# Autodesk Inventor assembly: EnsambleTuberiaVacio-Desfogue-Condensados
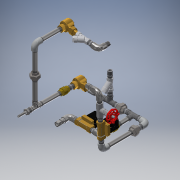
[picture p0: Inventor's stored thumbnail of the model, 180x180]
Saved by Autodesk Inventor 2017 (Build 210142000, 142)
## iProperties
Created: 2021-06-28
Part Number: EnsambleTuberiaVacio-Desfogue-Condensados
Document SubType Name: Assembly
Designer: USUARIO
Author: USUARIO
## Documents named in this file (17)
- D:\Laboratorio\Autoclave\Autoclave Horizontal\Con Precamara\2021\Autoclave 110L Biocacol OP2021110 #0045886XX\Modelo\Planos\EnsambleTuberiaVacio-Desfogue-Condensados.iam
- C:\Modelos 3D y DXF\Filtro en Y\Filtro Y 1-2'' Inox.ipt
- C:\Modelos 3D y DXF\Racores\B122 1-2x1-2.ipt
- C:\Modelos 3D y DXF\Racores\User Library-Tee_Class300.ipt
- C:\Modelos 3D y DXF\Racores\TRAMPA SPIRAX SARCO.ipt
- C:\Modelos 3D y DXF\Racores\Universal1-2.ipt
- C:\Modelos 3D y DXF\Racores\Niple 1-2x3.ipt
- C:\Modelos 3D y DXF\Racores\Check Valve 0.5.ipt
- C:\Modelos 3D y DXF\Racores\CodoCalle.iam
- C:\Modelos 3D y DXF\Danfoss EV210B\DANFOS EV225B.ipt
- C:\Modelos 3D y DXF\Racores\1-2-1-2-SwagelokCompany-3D-06-16-2021.ipt
- C:\Modelos 3D y DXF\Racores\User Library-codo a 90 de 1-2-Rosc.ipt
- C:\Modelos 3D y DXF\Racores\Niple 1-2x6.ipt
- D:\Laboratorio\Autoclave\Autoclave Horizontal\Con Precamara\2021\Autoclave 110L Biocacol OP2021110 #0045886XX\Modelo\UNION LISA 1-2.ipt
- C:\Modelos 3D y DXF\Racores\Niple 1-2x5.ipt
- C:\Modelos 3D y DXF\Racores\B3 1-2x1-2.ipt
- C:\Modelos 3D y DXF\Valvula de Globo\458513-15.iam
## Components (44 placed, 16 different names)
1. Filtro Y 1-2'' Inox:1
2. B122 1-2x1-2:1
3. B122 1-2x1-2:2
4. User Library-Tee_Class300:1
5. TRAMPA SPIRAX SARCO:1
6. B122 1-2x1-2:3
7. Universal1-2:1
8. B122 1-2x1-2:4
9. User Library-Tee_Class300:2
10. Niple 1-2x3:1
11. Check Valve 0.5:1
12. CodoCalle:1 [sub-assembly]
13. B122 1-2x1-2:5
14. DANFOS EV225B:1
15. CodoCalle:2 [sub-assembly]
16. 1-2-1-2-SwagelokCompany-3D-06-16-2021:1
17. User Library-codo a 90 de 1-2-Rosc:1
18. B122 1-2x1-2:6
19. User Library-codo a 90 de 1-2-Rosc:2
20. B122 1-2x1-2:7
21. Universal1-2:2
22. Niple 1-2x6:1
23. B122 1-2x1-2:8
24. DANFOS EV225B:2
25. B122 1-2x1-2:9
26. Check Valve 0.5:2
27. Filtro Y 1-2'' Inox:2
28. B122 1-2x1-2:10
29. CodoCalle:3 [sub-assembly]
30. TRAMPA SPIRAX SARCO:2
31. UNION LISA 1-2:1
32. Niple 1-2x3:2
33. Niple 1-2x5:1
34. Niple 1-2x5:2
35. User Library-codo a 90 de 1-2-Rosc:3
36. User Library-Tee_Class300:3
37. Universal1-2:3
38. Niple 1-2x5:3
39. Niple 1-2x5:4
40. B3 1-2x1-2:1
41. 458513-15:1 [sub-assembly]
42. B122 1-2x1-2:11
43. 1-2-1-2-SwagelokCompany-3D-06-16-2021:2
44. CodoCalle:4 [sub-assembly]
## Relationships (42: Insert 42)
- [Insert] (7 mm): Filtro Y 1-2'' Inox:1 ↔ B122 1-2x1-2:1
- [Insert] (9 mm): B122 1-2x1-2:2 ↔ User Library-Tee_Class300:1
- [Insert] (-7 mm): Filtro Y 1-2'' Inox:1 ↔ B122 1-2x1-2:2
- [Insert] (-9 mm): User Library-Tee_Class300:1 ↔ B122 1-2x1-2:3
- [Insert] (-12 mm): B122 1-2x1-2:3 ↔ Universal1-2:1
- [Insert] (-12 mm): Universal1-2:1 ↔ B122 1-2x1-2:4
- [Insert] (-12 mm): B122 1-2x1-2:4 ↔ User Library-Tee_Class300:2
- [Insert] (-12 mm): User Library-Tee_Class300:2 ↔ Niple 1-2x3:1
- [Insert] (7 mm): Niple 1-2x3:1 ↔ Check Valve 0.5:1
- [Insert] (-7 mm): Check Valve 0.5:1 ↔ CodoCalle:1
- [Insert] (-9 mm): B122 1-2x1-2:5 ↔ DANFOS EV225B:1
- [Insert] (-12 mm): CodoCalle:1 ↔ B122 1-2x1-2:5
- [Insert] (-12 mm): DANFOS EV225B:1 ↔ CodoCalle:2
- [Insert] (9 mm): CodoCalle:2 ↔ 1-2-1-2-SwagelokCompany-3D-06-16-2021:1
- [Insert] (-12 mm): User Library-Tee_Class300:2 ↔ B122 1-2x1-2:6
- [Insert] (-12 mm): User Library-codo a 90 de 1-2-Rosc:1 ↔ B122 1-2x1-2:6
- [Insert] (-12 mm): B122 1-2x1-2:7 ↔ Universal1-2:2
- [Insert] (-9 mm): User Library-codo a 90 de 1-2-Rosc:1 ↔ B122 1-2x1-2:7
- [Insert] (-12 mm): Universal1-2:2 ↔ Niple 1-2x6:1
- [Insert] (-12 mm): User Library-codo a 90 de 1-2-Rosc:2 ↔ Niple 1-2x6:1
- [Insert] (-9 mm): B122 1-2x1-2:8 ↔ DANFOS EV225B:2
- [Insert] (-9 mm): User Library-codo a 90 de 1-2-Rosc:2 ↔ B122 1-2x1-2:8
- [Insert] (-7 mm): B122 1-2x1-2:9 ↔ Check Valve 0.5:2
- [Insert] (-7 mm): TRAMPA SPIRAX SARCO:1 ↔ B122 1-2x1-2:9
- [Insert] (7 mm): Filtro Y 1-2'' Inox:2 ↔ B122 1-2x1-2:10
- [Insert] (-9 mm): B122 1-2x1-2:10 ↔ CodoCalle:3
- [Insert] (-9 mm): Filtro Y 1-2'' Inox:2 ↔ TRAMPA SPIRAX SARCO:2
- [Insert] (-12 mm): User Library-Tee_Class300:1 ↔ Niple 1-2x3:2
- [Insert] (-10 mm): UNION LISA 1-2:1 ↔ Niple 1-2x3:2
- [Insert] (-9 mm): TRAMPA SPIRAX SARCO:1 ↔ UNION LISA 1-2:1
- [Insert] (-9 mm): Check Valve 0.5:2 ↔ Niple 1-2x5:1
- [Insert] (-7 mm): TRAMPA SPIRAX SARCO:2 ↔ Niple 1-2x5:2
- [Insert] (-12 mm): Niple 1-2x5:2 ↔ User Library-codo a 90 de 1-2-Rosc:3
- [Insert] (-12 mm): Niple 1-2x5:1 ↔ User Library-Tee_Class300:3
- [Insert] (-12 mm): User Library-Tee_Class300:3 ↔ Niple 1-2x5:3
- [Insert] (-12 mm): Universal1-2:3 ↔ Niple 1-2x5:3
- [Insert] (-12 mm): Universal1-2:3 ↔ Niple 1-2x5:4
- [Insert] (-10 mm): User Library-Tee_Class300:3 ↔ B3 1-2x1-2:1
- [Insert] (-9 mm): 458513-15:1 ↔ B122 1-2x1-2:11
- [Insert] (-9 mm): DANFOS EV225B:2 ↔ B122 1-2x1-2:11
- [Insert] (-9 mm): 458513-15:1 ↔ CodoCalle:4
- [Insert] (9 mm): 1-2-1-2-SwagelokCompany-3D-06-16-2021:2 ↔ CodoCalle:4
## Named parameters: d52_d38_d9 = -9 mm, d54_d7 = -7 mm, d56_d26_d12 = 7 mm, d48_d32 = -12 mm, d38_d9 = -9 mm, d24_d39 = -12 mm, d25_d40 = -12 mm, d26_d41 = 9 mm, d28_d31 = -9 mm, d29_d32 = -12 mm, d30_d33 = -12 mm, d31_d34 = -12 mm, d32_d35 = -12 mm, d33_d36 = 7 mm, d34_d37 = -7 mm, d26_d12 = 7 mm, d28_d3 = 9 mm
